# Autodesk Inventor assembly: main
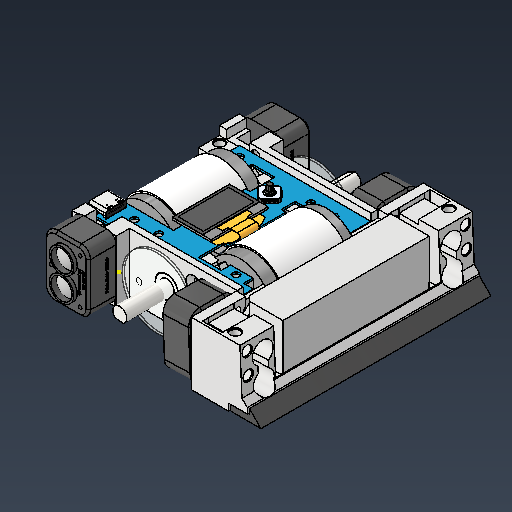
[picture p0: Inventor's stored thumbnail of the model, 512x512]
Saved by Autodesk Inventor 2026.2 (Build 302298010, 298A)
## iProperties
Created: 2026-03-09
Part Number: main
Document SubType Name: Assembly
Designer: szymo
Author: szymo
## Documents named in this file (17)
- D:\tech\robotyka\robots\evangelion-turbo\inventor-project\main.iam
- D:\tech\robotyka\robots\evangelion-turbo\inventor-project\drive-train.iam
- D:\tech\robotyka\robots\evangelion-turbo\inventor-project\LUNA.ipt
- D:\tech\robotyka\robots\evangelion-turbo\inventor-project\3s450mah.ipt
- D:\tech\robotyka\robots\evangelion-turbo\inventor-project\KTIR-Board.ipt
- D:\tech\robotyka\robots\evangelion-turbo\inventor-project\Left_gearbox.ipt
- D:\tech\robotyka\robots\evangelion-turbo\inventor-project\BearigHoldLeft.ipt
- D:\tech\robotyka\robots\evangelion-turbo\inventor-project\Right_gearbox.ipt
- D:\tech\robotyka\robots\evangelion-turbo\inventor-project\BearigHoldRight.ipt
- D:\tech\robotyka\robots\evangelion-turbo\inventor-project\LeftGearboxCover.ipt
- D:\tech\robotyka\robots\evangelion-turbo\inventor-project\plug.ipt
- D:\tech\robotyka\robots\evangelion-turbo\inventor-project\FonrtMount.ipt
- D:\tech\robotyka\robots\evangelion-turbo\inventor-project\RightGearboxCover.ipt
- D:\tech\robotyka\robots\evangelion-turbo\inventor-project\PCB_interface.ipt
- D:\tech\robotyka\robots\evangelion-turbo\inventor-project\TypC_port\TypC_port\TypC_port.ipt
- D:\tech\robotyka\robots\evangelion-turbo\inventor-project\0.96 oled\0.96 oled\0.96 oled.ipt
- D:\tech\robotyka\robots\evangelion-turbo\inventor-project\THMU 13 (SMD JOYSTICK)\THMU 13 (SMD JOYSTICK)\THMU 13 (SMD JOYSTICK).ipt
## Components (22 placed, 16 different names)
1. drive-train:1 [sub-assembly] — Flush:2, Flush:3, Flush:4, Mate:2, Mate:3, Tangent:1, Mate:9, Angle:3, Mate:13
2. 3s450mah:1 — Flush:8, Tangent:1, Flush:9
3. LUNA:2 — Mate:1, Mate:3, Angle:2, Mate:11, Flush:48, Flush:49, Flush:50
4. LUNA:1 — Flush:5, Mate:2, Angle:1, Mate:12
5. LUNA:3 — Flush:22, Flush:23, Mate:5, Mate:6
6. LUNA:4 — Flush:24, Flush:25, Flush:26, Mate:7
7. KTIR-Board:1 — Flush:10, Flush:11, Flush:13
8. KTIR-Board:2 — Mate:4, Flush:12, Flush:14
9. KTIR-Board:4 — Flush:17, Flush:27, Mate:6
10. KTIR-Board:5 — Flush:28, Flush:29, Mate:7
11. Left_gearbox:1 — Flush:33, Flush:35, Flush:37
12. BearigHoldLeft:1 — Flush:37, Flush:38
13. LeftGearboxCover:1 — Flush:43, Mate:13, Flush:46
14. Right_gearbox:1 — Flush:40, Flush:54
15. BearigHoldRight:1 — Flush:42
16. RightGearboxCover:1 — Flush:52
17. plug:1 — Flush:44, Mate:10, Flush:45
18. FonrtMount:1 — Flush:47, Flush:48, Flush:49, Flush:50
19. PCB_interface:1 — Flush:54, Mate:14
20. TypC_port:1
21. THMU 13 (SMD JOYSTICK):1
22. 0.96 oled:1 — Mate:14
## Relationships (60: Flush 43, Mate 13, Angle 3, Tangent 1)
- Flush:2 (0.65 mm): drive-train:1
- Flush:3 (-18.4 mm): drive-train:1
- Flush:4 (0.65 mm): drive-train:1
- Flush:5 (49.5 mm): LUNA:1
- Mate:1 (-49.5 mm): LUNA:2
- Mate:2 (18 mm): drive-train:1 ↔ LUNA:1
- Mate:3 (18 mm): drive-train:1 ↔ LUNA:2
- Angle:1 (-2 deg): LUNA:1
- Angle:2 (182 deg): LUNA:2
- Flush:8 (6.5 mm): 3s450mah:1
- Tangent:1 (0.65 mm): drive-train:1 ↔ 3s450mah:1
- Flush:9 (-31.5 mm): 3s450mah:1
- Flush:10 (-49 mm): KTIR-Board:1
- Mate:4 (-49 mm): KTIR-Board:2
- Flush:11 (0.13 mm): KTIR-Board:1
- Flush:12 (0.13 mm): KTIR-Board:2
- Flush:13 (65.5 mm): KTIR-Board:1
- Flush:14 (-65.5 mm): KTIR-Board:2
- Flush:17: KTIR-Board:4
- Flush:22: LUNA:3
- Flush:23 (1 mm): LUNA:3
- Mate:5 (-49.5 mm): LUNA:3
- Flush:24 (1 mm): LUNA:4
- Flush:25: LUNA:4
- Flush:26 (-49.5 mm): LUNA:4
- Flush:27 (0.5 mm): KTIR-Board:4
- Flush:28 (0.5 mm): KTIR-Board:5
- Flush:29: KTIR-Board:5
- Mate:6: LUNA:3 ↔ KTIR-Board:4
- Mate:7: LUNA:4 ↔ KTIR-Board:5
- Flush:32 (-19 mm)
- Flush:33: Left_gearbox:1
- Flush:34 (-23 mm)
- Flush:35: Left_gearbox:1
- Flush:36 (-18.4 mm)
- Flush:37: Left_gearbox:1 ↔ BearigHoldLeft:1
- Flush:38: BearigHoldLeft:1
- Flush:39 (19 mm)
- Flush:40: Right_gearbox:1
- Flush:41 (18.4 mm)
- Flush:42: BearigHoldRight:1
- Mate:9: drive-train:1
- Angle:3 (0 deg): drive-train:1
- Flush:43 (1.8 mm): LeftGearboxCover:1
- Flush:44 (81.9 mm): plug:1
- Mate:10 (-49.5 mm): plug:1
- Flush:45: plug:1
- Mate:11: LUNA:2
- Mate:12: LUNA:1
- Mate:13: drive-train:1 ↔ LeftGearboxCover:1
- Flush:46: LeftGearboxCover:1
- Flush:47: FonrtMount:1
- Flush:48: LUNA:2 ↔ FonrtMount:1
- Flush:49: LUNA:2 ↔ FonrtMount:1
- Flush:50: LUNA:2 ↔ FonrtMount:1
- Flush:51 (27.8 mm)
- Flush:52: RightGearboxCover:1
- Flush:53 (-29 mm)
- Flush:54: Right_gearbox:1 ↔ PCB_interface:1
- Mate:14: PCB_interface:1 ↔ 0.96 oled:1
